# Autodesk Inventor assembly: motor_35kg
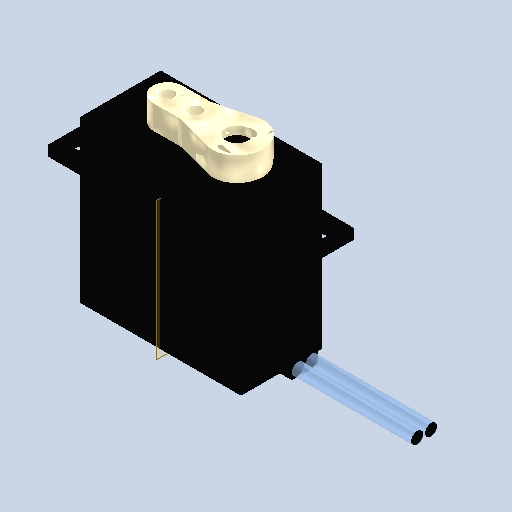
[picture p0: Inventor's stored thumbnail of the model, 512x512]
Saved by Autodesk Inventor 2025 (Build 290162000, 162)
## iProperties
Created: 2025-01-14
Part Number: motor_35kg
Document SubType Name: Assembly
Designer: Pauline Simonnet
Author: Pauline Simonnet
## Documents named in this file (3)
- C:\Users\Pauline Simonnet\Documents\ISAE SUPAERO\SupaeroMoon\MDRS\components\motor_35kg.iam
- C:\Users\Pauline Simonnet\Documents\ISAE SUPAERO\SupaeroMoon\MDRS\components\adaptator_35.ipt
- C:\Users\Pauline Simonnet\Documents\ISAE SUPAERO\SupaeroMoon\MDRS\components\motor_35kg.ipt
## Components (2 placed, 2 different names)
1. adaptator_35:1 — Mate:1, Mate:2
2. motor_35kg:1 — Mate:1, Mate:2
## Relationships (2: Mate 2)
- Mate:1: adaptator_35:1 ↔ motor_35kg:1
- Mate:2: adaptator_35:1 ↔ motor_35kg:1
